# Autodesk Inventor assembly: 160 mm lens
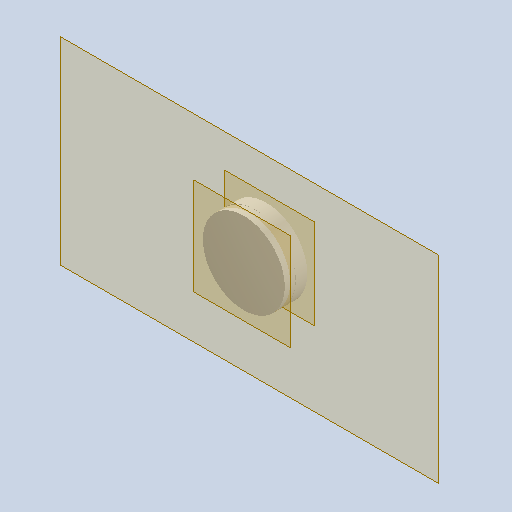
[picture p0: Inventor's stored thumbnail of the model, 512x512]
Saved by Autodesk Inventor 2026.1 (Build 301233000, 233)
## iProperties
Company: Unknown
Created: 2016-12-13
Part Number: 160 mm lens
Document SubType Name: Assembly
Designer: Julian
Sending System: HarmonyWare Translators
Preprocessor: HarmonyWare STEP v2.0.2
Title: C:\Users\dand\Desktop\temp\ExportCad\doublets\STEP_67331.STP
Author: Unknown
## Documents named in this file (3)
- C:\Users\user\Desktop\setup for publishing\160 mm lens.iam
- C:\Users\user\Desktop\setup for publishing\NONE.ipt
- C:\Users\user\Desktop\setup for publishing\NONE_1.ipt
## Components (2 placed, 2 different names)
1. NONE — Tangent:1, Mate:1, Angle:1
2. NONE_1 — Tangent:1, Mate:1, Tangent:2
## Relationships (5: Tangent 2, Mate 1, Angle 1, Flush 1)
- Tangent:1: NONE ↔ NONE_1
- Mate:1: NONE ↔ NONE_1
- Angle:1 (0 deg): NONE
- Tangent:2: NONE_1
- Flush:1 (-2.13 mm)
